# Autodesk Inventor assembly: Montagem_Lamina_Com_Suporte
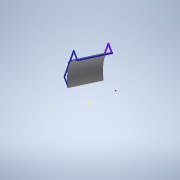
[picture p0: Inventor's stored thumbnail of the model, 180x180]
Saved by Autodesk Inventor 2022 (Build 260153000, 153)
## iProperties
Created: 2016-02-21
Part Number: Montagem_Lamina_Com_Suporte
Document SubType Name: Assembly
Designer: Everton
Author: Everton
## Documents named in this file (7)
- C:\Users\Alison\Documents\TCC\Peças e desenho no inventor - TCC\Peças\Montagem_Lamina_Com_Suporte.iam
- C:\Users\Alison\Documents\TCC\Desenhos e Montagem\desenhos e montagems inventor 15\SUPORTE_LAMINA_COM_BASE.ipt
- C:\Users\Alison\Documents\TCC\Desenhos e Montagem\desenhos e montagems inventor 15\BASE_FUNDO_SUPORTE_LAMINA.ipt
- C:\Users\Alison\Documents\TCC\Desenhos e Montagem\desenhos e montagems inventor 15\CHAPA_CALÇO_CURVADA.ipt
- C:\Users\Alison\Documents\TCC\Desenhos e Montagem\desenhos e montagems inventor 15\MANCAL_FIXO.ipt
- C:\Users\Alison\Documents\TCC\Desenhos e Montagem\desenhos e montagems inventor 15\BUCHA.ipt
- C:\Users\Alison\Documents\TCC\Desenhos e Montagem\desenhos e montagems inventor 15\CHAPA_INOX.ipt
## Components (10 placed, 6 different names)
1. SUPORTE_LAMINA_COM_BASE:1 — Flush:1, Flush:2, Flush:3, Flush:4, Flush:5, Flush:6, Mate:1, Mate:18, Coincidente:26, Tangente:4, Alinhado:7, Tangente:6
2. BASE_FUNDO_SUPORTE_LAMINA:1 — Flush:1, Flush:2, Flush:3, Mate:2, Coincidente:20, Coincidente:24, Coincidente:25
3. CHAPA_CALÇO_CURVADA:1 — Flush:4, Flush:5, Flush:6, Mate:1, Mate:13, Mate:14, Mate:17
4. MANCAL_FIXO:1 — Mate:2, Coincidente:26, Coincidente:27, Tangente:4, Tangente:5
5. BUCHA:1 — Coincidente:27, Tangente:5
6. MANCAL_FIXO:2 — Coincidente:20, Coincidente:22, Coincidente:24, Coincidente:25, Tangente:3
7. BUCHA:2 — Coincidente:22, Tangente:3
8. CHAPA_CALÇO_CURVADA:2 — Mate:13, Mate:14, Mate:15, Mate:16, Mate:17
9. CHAPA_CALÇO_CURVADA:3 — Mate:15, Mate:16, Mate:18
10. CHAPA_INOX:1 — Alinhado:7, Tangente:6
## Relationships (25: Mate 14, Flush 7, Tangent 4)
- Flush:1: SUPORTE_LAMINA_COM_BASE:1 ↔ BASE_FUNDO_SUPORTE_LAMINA:1
- Flush:2: SUPORTE_LAMINA_COM_BASE:1 ↔ BASE_FUNDO_SUPORTE_LAMINA:1
- Flush:3: SUPORTE_LAMINA_COM_BASE:1 ↔ BASE_FUNDO_SUPORTE_LAMINA:1
- Flush:4: SUPORTE_LAMINA_COM_BASE:1 ↔ CHAPA_CALÇO_CURVADA:1
- Flush:5: SUPORTE_LAMINA_COM_BASE:1 ↔ CHAPA_CALÇO_CURVADA:1
- Flush:6: SUPORTE_LAMINA_COM_BASE:1 ↔ CHAPA_CALÇO_CURVADA:1
- Mate:1: SUPORTE_LAMINA_COM_BASE:1 ↔ CHAPA_CALÇO_CURVADA:1
- Mate:2: BASE_FUNDO_SUPORTE_LAMINA:1 ↔ MANCAL_FIXO:1
- Mate:13: CHAPA_CALÇO_CURVADA:1 ↔ CHAPA_CALÇO_CURVADA:2
- Mate:14: CHAPA_CALÇO_CURVADA:1 ↔ CHAPA_CALÇO_CURVADA:2
- Mate:15: CHAPA_CALÇO_CURVADA:2 ↔ CHAPA_CALÇO_CURVADA:3
- Mate:16: CHAPA_CALÇO_CURVADA:2 ↔ CHAPA_CALÇO_CURVADA:3
- Mate:17 (315 mm): CHAPA_CALÇO_CURVADA:1 ↔ CHAPA_CALÇO_CURVADA:2
- Mate:18 (315 mm): SUPORTE_LAMINA_COM_BASE:1 ↔ CHAPA_CALÇO_CURVADA:3
- Coincidente:20 [Mate]: BASE_FUNDO_SUPORTE_LAMINA:1 ↔ MANCAL_FIXO:2
- Coincidente:22 [Mate]: MANCAL_FIXO:2 ↔ BUCHA:2
- Coincidente:24 [Mate]: BASE_FUNDO_SUPORTE_LAMINA:1 ↔ MANCAL_FIXO:2
- Coincidente:25 [Mate]: BASE_FUNDO_SUPORTE_LAMINA:1 ↔ MANCAL_FIXO:2
- Tangente:3: MANCAL_FIXO:2 ↔ BUCHA:2
- Coincidente:26 [Mate]: SUPORTE_LAMINA_COM_BASE:1 ↔ MANCAL_FIXO:1
- Coincidente:27 [Mate]: MANCAL_FIXO:1 ↔ BUCHA:1
- Tangente:4: SUPORTE_LAMINA_COM_BASE:1 ↔ MANCAL_FIXO:1
- Tangente:5: MANCAL_FIXO:1 ↔ BUCHA:1
- Alinhado:7 [Flush]: SUPORTE_LAMINA_COM_BASE:1 ↔ CHAPA_INOX:1
- Tangente:6 (3 mm): SUPORTE_LAMINA_COM_BASE:1 ↔ CHAPA_INOX:1
